# Autodesk Inventor assembly: printer
(part 2 of 2)
- Insert:42: CSN 02 1702 B B 4,3:138 ↔ ISO 4762 M4 x 20:73
- Mate:235: ISO 4762 M4 x 20:70 ↔ DIN EN ISO 7040 M4:58
- Mate:236: CSN 02 1702 B B 4,3:145 ↔ DIN EN ISO 7040 M4:58
- Mate:237: ISO 4762 M4 x 20:71 ↔ DIN EN ISO 7040 M4:59
- Mate:238: CSN 02 1702 B B 4,3:144 ↔ DIN EN ISO 7040 M4:59
- Mate:239: ISO 4762 M4 x 20:72 ↔ DIN EN ISO 7040 M4:60
- Mate:240: CSN 02 1702 B B 4,3:137 ↔ DIN EN ISO 7040 M4:60
- Mate:241: ISO 4762 M4 x 20:68 ↔ DIN EN ISO 7040 M4:61
- Mate:242: CSN 02 1702 B B 4,3:143 ↔ DIN EN ISO 7040 M4:61
- Mate:243: ISO 4762 M4 x 20:69 ↔ DIN EN ISO 7040 M4:62
- Mate:244: CSN 02 1702 B B 4,3:146 ↔ DIN EN ISO 7040 M4:62
- Mate:245: ISO 4762 M4 x 20:73 ↔ DIN EN ISO 7040 M4:63
- Mate:246: CSN 02 1702 B B 4,3:133 ↔ DIN EN ISO 7040 M4:63
- Mate:247: ISO 4762 M4 x 20:67 ↔ DIN EN ISO 7040 M4:64
- Mate:248: CSN 02 1702 B B 4,3:136 ↔ DIN EN ISO 7040 M4:64
- Mate:249: CSN 02 1702 B B 4,3:149 ↔ ISO 4762 M4 x 20:74
- Insert:43: CSN 02 1702 B B 4,3:150 ↔ ISO 4762 M4 x 20:74
- Mate:250: CSN 02 1702 B B 4,3:148 ↔ ISO 4762 M4 x 20:75
- Insert:44: CSN 02 1702 B B 4,3:147 ↔ ISO 4762 M4 x 20:75
- Mate:251: ISO 4762 M4 x 20:75 ↔ DIN EN ISO 7040 M4:65
- Mate:252: CSN 02 1702 B B 4,3:148 ↔ DIN EN ISO 7040 M4:65
- Mate:253: ISO 4762 M4 x 20:74 ↔ DIN EN ISO 7040 M4:66
- Mate:254: CSN 02 1702 B B 4,3:149 ↔ DIN EN ISO 7040 M4:66
- Insert:45: CSN 02 1702 B B 3,2:6 ↔ ISO 4762 M3 x 16:5
- Insert:46: CSN 02 1702 B B 3,2:8 ↔ ISO 4762 M3 x 16:6
- Insert:47: CSN 02 1702 B B 3,2:7 ↔ ISO 4762 M3 x 16:7
- Insert:48: CSN 02 1702 B B 3,2:5 ↔ ISO 4762 M3 x 16:8
- Mate:255: back:1 ↔ PC Fan:1
- Mate:256: back:1 ↔ PC Fan:1
- Mate:257: back:1 ↔ PC Fan:1
- Mate:258 (3 mm): back:1 ↔ User Library-Fan Guard:1
- Mate:259: y_carriage_belt_iddler:2 ↔ y_carriage_belt_iddler_holder:1
- Mate:260: y_carriage_belt_iddler:2 ↔ y_carriage_belt_iddler_holder:1
- Mate:261: y_carriage_belt_iddler:2 ↔ y_carriage_belt_iddler_holder:1
- Mate:262: y_carriage_belt_iddler:1 ↔ y_carriage_belt_iddler_holder:1
- Mate:263: y_carriage_belt_iddler:1 ↔ y_carriage_belt_iddler_holder:1
- Mate:264: y_carriage_belt_iddler:1 ↔ y_carriage_belt_iddler_holder:1
- Mate:265: 608RS:1 ↔ belt_guide:1
- Mate:266: 608RS:1 ↔ belt_guide:1
- Mate:267: belt_guide:1 ↔ belt_guide:2
- Mate:268: belt_guide:1 ↔ belt_guide:2
- Mate:269: 608RS:1 ↔ belt_guide:2
- Mate:270: CSN 02 1702 B B 8,4:5 ↔ CSN 02 1702 B B 8,4:6
- Mate:271: CSN 02 1702 B B 8,4:5 ↔ CSN 02 1702 B B 8,4:6
- Mate:272: CSN 02 1702 B B 8,4:3 ↔ CSN 02 1702 B B 8,4:4
- Mate:273: CSN 02 1702 B B 8,4:3 ↔ CSN 02 1702 B B 8,4:4
- Mate:274: 608RS:1 ↔ CSN 02 1702 B B 8,4:4
- Mate:275: 608RS:1 ↔ CSN 02 1702 B B 8,4:4
- Mate:276: 608RS:1 ↔ CSN 02 1702 B B 8,4:5
- Mate:277: 608RS:1 ↔ CSN 02 1702 B B 8,4:5
- Mate:278: y_carriage_belt_iddler:1 ↔ CSN 02 1702 B B 8,4:6
- Mate:279: y_carriage_belt_iddler:2 ↔ 608RS:1
- Mate:280: y_carriage_belt_iddler:2 ↔ CSN 02 1702 B B 8,4:1
- Mate:281: y_carriage_belt_iddler:2 ↔ CSN 02 1702 B B 8,4:1
- Mate:282: y_carriage_belt_iddler:1 ↔ CSN 02 1702 B B 8,4:2
- Mate:283: y_carriage_belt_iddler:1 ↔ CSN 02 1702 B B 8,4:2
- Insert:49: CSN 02 1702 B B 8,4:2 ↔ ISO 4762 M8 x 40:1
- Mate:284: CSN 02 1702 B B 8,4:1 ↔ DIN EN ISO 7040 M8:1
- Mate:285: ISO 4762 M8 x 40:1 ↔ DIN EN ISO 7040 M8:1
- Mate:286: back:1 ↔ y_carriage_belt_iddler:2
- Mate:287: back:1 ↔ y_carriage_belt_iddler:2
- Mate:288: back:1 ↔ y_carriage_belt_iddler:1
- Mate:289: back:1 ↔ CSN 02 1702 B B 4,3:152
- Mate:290: back:1 ↔ CSN 02 1702 B B 4,3:153
- Mate:291: back:1 ↔ CSN 02 1702 B B 4,3:153
- Mate:292: back:1 ↔ CSN 02 1702 B B 4,3:152
- Insert:50: CSN 02 1702 B B 4,3:152 ↔ ISO 4762 M4 x 30:1
- Insert:51: CSN 02 1702 B B 4,3:153 ↔ ISO 4762 M4 x 30:2
- Mate:293: y_carriage_belt_iddler_holder:1 ↔ CSN 02 1702 B B 4,3:154
- Mate:294: y_carriage_belt_iddler_holder:1 ↔ CSN 02 1702 B B 4,3:151
- Mate:295: CSN 02 1702 B B 4,3:151 ↔ ISO 4762 M4 x 30:2
- Mate:296: CSN 02 1702 B B 4,3:154 ↔ ISO 4762 M4 x 30:1
- Mate:297: CSN 02 1702 B B 4,3:151 ↔ DIN EN ISO 7040 M4:68
- Mate:298: ISO 4762 M4 x 30:2 ↔ DIN EN ISO 7040 M4:68
- Mate:299: CSN 02 1702 B B 4,3:154 ↔ DIN EN ISO 7040 M4:67
- Mate:300: ISO 4762 M4 x 30:1 ↔ DIN EN ISO 7040 M4:67
- Mate:301: y_motor_mount:1 ↔ y_motor_mount_brace:1
- Mate:302: y_motor_mount:1 ↔ y_motor_mount_brace:1
- Mate:303: y_motor_mount:1 ↔ y_motor_mount_brace:1
- Mate:304: front:1 ↔ y_motor_mount:1
- Mate:305: front:1 ↔ y_motor_mount_brace:1
- Mate:306: front:1 ↔ y_motor_mount:1
- Mate:307: front:1 ↔ CSN 02 1702 B B 4,3:159
- Mate:308: front:1 ↔ CSN 02 1702 B B 4,3:160
- Mate:309: front:1 ↔ CSN 02 1702 B B 4,3:160
- Mate:310: front:1 ↔ CSN 02 1702 B B 4,3:159
- Mate:311: y_motor_mount:1 ↔ CSN 02 1702 B B 4,3:157
- Mate:312: y_motor_mount:1 ↔ CSN 02 1702 B B 4,3:157
- Insert:52: CSN 02 1702 B B 4,3:160 ↔ ISO 4762 M4 x 20:78
- Insert:53: CSN 02 1702 B B 4,3:159 ↔ ISO 4762 M4 x 20:77
- Insert:54: CSN 02 1702 B B 4,3:157 ↔ ISO 4762 M4 x 20:76
- Mate:313: y_motor_mount_brace:1 ↔ CSN 02 1702 B B 4,3:158
- Mate:314: CSN 02 1702 B B 4,3:158 ↔ ISO 4762 M4 x 20:78
- Mate:315: y_motor_mount_brace:1 ↔ CSN 02 1702 B B 4,3:155
- Mate:316: CSN 02 1702 B B 4,3:155 ↔ ISO 4762 M4 x 20:76
- Mate:317: y_motor_mount:1 ↔ CSN 02 1702 B B 4,3:156
- Mate:318: CSN 02 1702 B B 4,3:156 ↔ ISO 4762 M4 x 20:77
- Mate:319: CSN 02 1702 B B 4,3:156 ↔ DIN EN ISO 7040 M4:70
- Mate:320: ISO 4762 M4 x 20:77 ↔ DIN EN ISO 7040 M4:70
- Mate:321: CSN 02 1702 B B 4,3:158 ↔ DIN EN ISO 7040 M4:69
- Mate:322: ISO 4762 M4 x 20:78 ↔ DIN EN ISO 7040 M4:69
- Mate:323: CSN 02 1702 B B 4,3:155 ↔ DIN EN ISO 7040 M4:71
- Mate:324: ISO 4762 M4 x 20:76 ↔ DIN EN ISO 7040 M4:71
- Mate:325: motor_spacer:1 ↔ NEMA 17 with T5 Pulley:1
- Mate:326: motor_spacer:1 ↔ NEMA 17 with T5 Pulley:1
- Mate:327: motor_spacer:1 ↔ NEMA 17 with T5 Pulley:1
- Mate:328: y_motor_mount:1 ↔ motor_spacer:1
- Tangent:1: y_motor_mount:1 ↔ motor_spacer:1
- Tangent:2: y_motor_mount:1 ↔ motor_spacer:1
- Mate:329: y_motor_mount:1 ↔ CSN 02 1702 B B 3,2:12
- Mate:330: y_motor_mount:1 ↔ CSN 02 1702 B B 3,2:11
- Mate:331: y_motor_mount:1 ↔ CSN 02 1702 B B 3,2:9
- Mate:332: y_motor_mount:1 ↔ CSN 02 1702 B B 3,2:10
- Insert:55: CSN 02 1702 B B 3,2:12 ↔ ISO 4762 M3 x 16:12
- Insert:56: CSN 02 1702 B B 3,2:11 ↔ ISO 4762 M3 x 16:11
- Insert:57: CSN 02 1702 B B 3,2:9 ↔ ISO 4762 M3 x 16:10
- Insert:58: CSN 02 1702 B B 3,2:10 ↔ ISO 4762 M3 x 16:9
- Mate:333: motor_spacer:1 ↔ ISO 4762 M3 x 16:12
- Mate:334: motor_spacer:1 ↔ ISO 4762 M3 x 16:11
- Mate:335: motor_spacer:1 ↔ ISO 4762 M3 x 16:9
- Mate:336: motor_spacer:1 ↔ ISO 4762 M3 x 16:10
- Mate:337: y_axis_rod:2 ↔ y_carryage:1
- Mate:338: y_axis_rod:1 ↔ y_carryage:1
- Mate:339: z_axis_rod:2 ↔ x_axis:1
- Mate:340: z_axis_rod:1 ↔ x_axis:1
- Mate:341: brace_right:1 ↔ CSN 02 1702 B B 4,3:161
- Mate:342: brace_right:1 ↔ CSN 02 1702 B B 4,3:161
- Insert:59: CSN 02 1702 B B 4,3:161 ↔ ISO 4762 M4 x 20:79
- Mate:343: frame_brace_top:1 ↔ CSN 02 1702 B B 4,3:162
- Mate:344: CSN 02 1702 B B 4,3:162 ↔ ISO 4762 M4 x 20:79
- Mate:345: CSN 02 1702 B B 4,3:162 ↔ DIN EN ISO 7040 M4:72
- Mate:346: ISO 4762 M4 x 20:79 ↔ DIN EN ISO 7040 M4:72
- Mate:347: CSN 02 1702 B B 4,3:164 ↔ ISO 4762 M4 x 20:80
- Insert:60: CSN 02 1702 B B 4,3:163 ↔ ISO 4762 M4 x 20:80
- Mate:348: ISO 4762 M4 x 20:80 ↔ DIN EN ISO 7040 M4:73
- Mate:349: CSN 02 1702 B B 4,3:164 ↔ DIN EN ISO 7040 M4:73
- Mate:350: z_axis_top_cap:2 ↔ CSN 02 1702 B B 4,3:172
- Mate:351: z_axis_top_cap:2 ↔ CSN 02 1702 B B 4,3:174
- Mate:352: z_axis_top_cap:2 ↔ CSN 02 1702 B B 4,3:174
- Mate:353: z_axis_top_cap:2 ↔ CSN 02 1702 B B 4,3:172
- Mate:354: z_axis_top:2 ↔ CSN 02 1702 B B 4,3:173
- Mate:355: z_axis_top:2 ↔ CSN 02 1702 B B 4,3:171
- Mate:356: z_axis_top:2 ↔ CSN 02 1702 B B 4,3:170
- Mate:357: z_axis_top:2 ↔ CSN 02 1702 B B 4,3:170
- Mate:358: z_axis_top:2 ↔ CSN 02 1702 B B 4,3:173
- Mate:359: z_axis_top:2 ↔ CSN 02 1702 B B 4,3:171
- Insert:61: CSN 02 1702 B B 4,3:170 ↔ ISO 4762 M4 x 20:81
- Insert:62: CSN 02 1702 B B 4,3:171 ↔ ISO 4762 M4 x 20:82
- Insert:63: CSN 02 1702 B B 4,3:173 ↔ ISO 4762 M4 x 20:83
- Insert:64: CSN 02 1702 B B 4,3:174 ↔ ISO 4762 M4 x 20:84
- Insert:65: CSN 02 1702 B B 4,3:172 ↔ ISO 4762 M4 x 20:85
- Mate:360: brace_right:1 ↔ CSN 02 1702 B B 4,3:169
- Mate:361: CSN 02 1702 B B 4,3:169 ↔ ISO 4762 M4 x 20:81
- Mate:362: frame:1 ↔ CSN 02 1702 B B 4,3:165
- Mate:363: CSN 02 1702 B B 4,3:165 ↔ ISO 4762 M4 x 20:83
- Mate:364: frame:1 ↔ CSN 02 1702 B B 4,3:166
- Mate:365: CSN 02 1702 B B 4,3:166 ↔ ISO 4762 M4 x 20:82
- Mate:366: z_axis_top:2 ↔ CSN 02 1702 B B 4,3:167
- Mate:367: CSN 02 1702 B B 4,3:167 ↔ ISO 4762 M4 x 20:84
- Mate:368: z_axis_top:2 ↔ CSN 02 1702 B B 4,3:168
- Mate:369: CSN 02 1702 B B 4,3:169 ↔ DIN EN ISO 7040 M4:78
- Mate:370: ISO 4762 M4 x 20:81 ↔ DIN EN ISO 7040 M4:78
- Mate:371: CSN 02 1702 B B 4,3:166 ↔ DIN EN ISO 7040 M4:77
- Mate:372: ISO 4762 M4 x 20:82 ↔ DIN EN ISO 7040 M4:77
- Mate:373: CSN 02 1702 B B 4,3:165 ↔ DIN EN ISO 7040 M4:76
- Mate:374: ISO 4762 M4 x 20:83 ↔ DIN EN ISO 7040 M4:76
- Mate:375: CSN 02 1702 B B 4,3:167 ↔ DIN EN ISO 7040 M4:75
- Mate:376: ISO 4762 M4 x 20:84 ↔ DIN EN ISO 7040 M4:75
- Mate:377: CSN 02 1702 B B 4,3:168 ↔ DIN EN ISO 7040 M4:74
- Mate:378: CSN 02 1702 B B 4,3:168 ↔ ISO 4762 M4 x 20:85
- Mate:379: ISO 4762 M4 x 20:85 ↔ DIN EN ISO 7040 M4:74
- Mate:380: CSN 02 1702 B B 4,3:179 ↔ ISO 4762 M4 x 20:86
- Insert:66: CSN 02 1702 B B 4,3:180 ↔ ISO 4762 M4 x 20:86
- Mate:381: CSN 02 1702 B B 4,3:176 ↔ ISO 4762 M4 x 20:87
- Insert:67: CSN 02 1702 B B 4,3:181 ↔ ISO 4762 M4 x 20:87
- Mate:382: CSN 02 1702 B B 4,3:175 ↔ ISO 4762 M4 x 20:88
- Insert:68: CSN 02 1702 B B 4,3:183 ↔ ISO 4762 M4 x 20:88
- Mate:383: CSN 02 1702 B B 4,3:177 ↔ ISO 4762 M4 x 20:89
- Insert:69: CSN 02 1702 B B 4,3:184 ↔ ISO 4762 M4 x 20:89
- Mate:384: CSN 02 1702 B B 4,3:178 ↔ ISO 4762 M4 x 20:90
- Insert:70: CSN 02 1702 B B 4,3:182 ↔ ISO 4762 M4 x 20:90
- Mate:385: ISO 4762 M4 x 20:90 ↔ DIN EN ISO 7040 M4:79
- Mate:386: CSN 02 1702 B B 4,3:178 ↔ DIN EN ISO 7040 M4:79
- Mate:387: ISO 4762 M4 x 20:89 ↔ DIN EN ISO 7040 M4:80
- Mate:388: CSN 02 1702 B B 4,3:177 ↔ DIN EN ISO 7040 M4:80
- Mate:389: ISO 4762 M4 x 20:88 ↔ DIN EN ISO 7040 M4:81
- Mate:390: CSN 02 1702 B B 4,3:175 ↔ DIN EN ISO 7040 M4:81
- Mate:391: ISO 4762 M4 x 20:87 ↔ DIN EN ISO 7040 M4:82
- Mate:392: CSN 02 1702 B B 4,3:176 ↔ DIN EN ISO 7040 M4:82
- Mate:393: ISO 4762 M4 x 20:86 ↔ DIN EN ISO 7040 M4:83
- Mate:394: CSN 02 1702 B B 4,3:179 ↔ DIN EN ISO 7040 M4:83
